# Autodesk Inventor assembly: large ball knocker metal_MIR
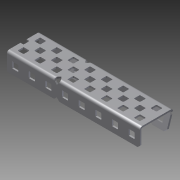
[picture p0: Inventor's stored thumbnail of the model, 180x180]
Saved by Autodesk Inventor 2014 SP1 (Build 180222100, 222)
## iProperties
Created: 2014-03-20
Part Number: large ball knocker metal_MIR
Document SubType Name: Assembly
Designer: Ryan
Author: Ryan
## Documents named in this file (3)
- C:\Users\Ryan\Desktop\sw\toss up 5th A bot\tower\large ball knocker metal_MIR.iam
- C:\Users\Ryan\Desktop\sw\lib\Aperture VEX CAD Library\Metal\C Channel\2 x 8 holes for large ball knockers_MIR.ipt
- C:\Users\Ryan\Desktop\sw\lib\Aperture VEX CAD Library\Metal\Custom 1 bar\1x1.ipt
## Components (3 placed, 2 different names)
1. 2 x 8 holes for large ball knockers_MIR:1 — Angle:1, Mate:2, Mate:1, Mate:4, Mate:3
2. 1x1:1 — Angle:1, Mate:2, Mate:1, Flush:1
3. 1x1:2 — Flush:1, Mate:4, Mate:3
## Relationships (6: Mate 4, Angle 1, Flush 1)
- Angle:1 (18.03 deg): 2 x 8 holes for large ball knockers_MIR:1 ↔ 1x1:1
- Mate:2: 2 x 8 holes for large ball knockers_MIR:1 ↔ 1x1:1
- Mate:1: 2 x 8 holes for large ball knockers_MIR:1 ↔ 1x1:1
- Flush:1: 1x1:1 ↔ 1x1:2
- Mate:4: 2 x 8 holes for large ball knockers_MIR:1 ↔ 1x1:2
- Mate:3: 2 x 8 holes for large ball knockers_MIR:1 ↔ 1x1:2
